# Autodesk Inventor assembly: Arm 2.0 Assembly
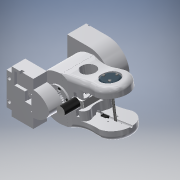
[picture p0: Inventor's stored thumbnail of the model, 180x180]
Saved by Autodesk Inventor 2017 (Build 210142000, 142)
## iProperties
Created: 2017-09-28
Part Number: Arm 2.0 Assembly
Document SubType Name: Assembly
Designer: Zach
Author: Zach
## Documents named in this file (28)
- C:\Users\Dell\Documents\GitHub\tr1\src\Body\Arm Assembly\Shoulder Assembly\Shoulder Assembly, Left.iam
- C:\Users\Dell\Documents\GitHub\tr1\src\Body\Arm Assembly\Shoulder Assembly\Steel Rod 8mm x 135mm.ipt
- C:\Users\Dell\Documents\GitHub\tr1\lib\22x8x8mm Bearing.ipt
- C:\Users\Dell\Documents\GitHub\tr1\src\Body\Arm Assembly\Shoulder Assembly\AA004.ipt
- C:\Users\Dell\Documents\GitHub\tr1\lib\QS12MM250\QS12MM250.ipt
- C:\Users\Dell\Documents\GitHub\tr1\src\Body\Arm Assembly\Shoulder Assembly\AA013.ipt
- C:\Users\Dell\Documents\GitHub\tr1\lib\12V DC Motor 378-1.ipt
- C:\Users\Dell\Documents\GitHub\tr1\lib\Content Center Files\R2017\en-US\ISO 4017(1)\ISO 4017 - M5 x 20 - ISO.ipt
- C:\Users\Dell\Documents\GitHub\tr1\lib\8mm Hub.ipt
- C:\Users\Dell\Documents\GitHub\tr1\src\Body\Arm Assembly\Arm Assembly\Design Accelerator\Spur Gears5.iam
- C:\Users\Dell\Documents\GitHub\tr1\lib\4mm mounting hub.ipt
- C:\Users\Dell\Documents\GitHub\tr1\lib\6201RS\6201RS.ipt
- C:\Users\Dell\Documents\GitHub\tr1\lib\U51105\U51105.ipt
- C:\Users\Dell\Documents\GitHub\tr1\src\Body\Arm Assembly\Shoulder Assembly\AA005b.ipt
- C:\Users\Dell\Documents\GitHub\tr1\src\Body\Arm Assembly\Shoulder Assembly\AA006b.ipt
- C:\Users\Dell\Documents\GitHub\tr1\src\Body\Arm Assembly\Arm Assembly\Design Accelerator\Spur Gears8.iam
- C:\Users\Dell\Documents\GitHub\tr1\src\Body\Arm Assembly\Arm Assembly\Design Accelerator\Spur Gears11.iam
- C:\Users\Dell\Documents\GitHub\tr1\lib\Content Center Files\R2017\en-US\ISO 7045  H\ISO 7045 - M3 x 8 - 4.8 - H - ISO.ipt
- C:\Users\Dell\Documents\GitHub\tr1\lib\Content Center Files\R2017\en-US\ISO 4018\ISO 4018 - M5 x 25.ipt
- C:\Users\Dell\Documents\GitHub\tr1\lib\Content Center Files\R2017\en-US\ISO 7045  H\ISO 7045 - M3 x 12 - 4.8 - H - ISO.ipt
- C:\Users\Dell\Documents\GitHub\tr1\lib\Content Center Files\R2017\en-US\ISO 4762(2)\ISO 4762 - M4 x 10ISO.ipt
- C:\Users\Dell\Documents\GitHub\tr1\lib\6mm Mounting Hub.ipt
- C:\Users\Dell\Documents\GitHub\tr1\lib\TSINY TS-42GZ495.ipt
- C:\Users\Dell\Documents\GitHub\tr1\lib\EMS22XXX-D28-LSX.ipt
- C:\Users\Dell\Documents\GitHub\tr1\src\Body\Arm Assembly\Shoulder Assembly\AA053.ipt
- C:\Users\Dell\Documents\GitHub\tr1\src\Body\Arm Assembly\Shoulder Assembly\AA057.ipt
- C:\Users\Dell\Documents\GitHub\tr1\src\Body\Arm Assembly\Shoulder Assembly\AASG02a.ipt
- C:\Users\Dell\Documents\GitHub\tr1\src\Body\Arm Assembly\Shoulder Assembly\AA001l.ipt
## Components (63 placed, 27 different names)
1. AA001l:1 — Mate:1312, Mate:1313, Mate:1314, Mate:1316, Mate:1317, Mate:1319, Mate:1320, Mate:1321, Mate:1322, Mate:1323, Mate:1324, Mate:1325, Mate:1326, Mate:1327, Mate:1328, Mate:1331, Mate:1332, Angle:18
2. AA004:1 — Mate:23, Mate:345, Mate:347, Mate:350, Mate:357, Mate:590
3. AA005b:1 — Mate:537, Mate:538, Mate:539, Mate:541, Mate:542, Mate:543, Mate:806, Mate:807, Mate:808, Mate:809, Mate:838, Mate:909, Mate:910
4. AA006b:1 — Mate:594, Mate:598, Mate:599, Mate:609, Mate:802, Mate:803, Mate:804, Mate:805, Mate:838, Mate:1088, Mate:1089, Angle:17, Mate:1233
5. AA013:2 — Mate:142, Mate:143, Mate:144, Mate:145, Mate:146, Mate:147, Mate:1281, Mate:1317, Mate:1318
6. AA053:3 — Mate:1331, Mate:1332, Angle:18
7. AA057:1 — Mate:1293, Mate:1295, Mate:1296, Mate:1297, Mate:1323
8. 22x8x8mm Bearing:1 — Mate:433, Mate:1316, Mate:1318
9. 22x8x8mm Bearing:2 — Mate:437
10. QS12MM250:1 — Mate:23, Mate:344, Mate:346, Mate:348, Mate:354, Mate:537, Mate:594, Mate:597, Mate:1230
11. Steel Rod 8mm x 140mm:1 — Mate:433, Mate:437, Mate:575, Flush:35
12. TSINY TS-42GZ495:1 — Mate:1293, Mate:1324, Mate:1325, Mate:1326, Mate:1329, Mate:1330
13. 12V DC Motor 378-1:6 — Mate:340, Mate:342, Mate:538, Mate:539, Mate:540, Mate:543, Mate:907, Mate:908
14. 6201RS:1 — Mate:346, Mate:347
15. 6201RS:2 — Mate:357, Mate:597
16. U51105:1 — Mate:348, Mate:349, Mate:542
17. U51105:2 — Mate:354, Mate:608, Mate:609, Mate:600
18. 6mm Mounting Hub:5 — Mate:1177, Mate:1178, Mate:1179, Mate:1300, Mate:1301, Mate:1302, Mate:1303, Mate:1304, Mate:1305
19. 6mm Mounting Hub:2 — Mate:1090, Mate:1091
20. 8mm Hub:4 — Mate:580, Mate:582, Flush:35, Mate:1315
21. 4mm mounting hub:1 — Mate:340, Mate:540, Mate:541, Mate:887
22. EMS22XXX-D28-LSX:1 — Mate:1088, Mate:1089, Angle:17, Mate:1090, Mate:1091, Mate:1182, Mate:1232
23. EMS22XXX-D28-LSX:2 — Mate:1177, Mate:1180, Mate:1319, Mate:1320
24. AASG01 [sub-assembly] — Mate:342, Mate:344, Mate:345, Mate:349, Mate:350, Mate:810, Mate:811, Mate:812, Mate:813, Mate:814, Mate:815, Mate:816, Mate:817, Mate:818, Mate:819, Mate:820, Mate:821, Mate:887, Mate:888, Mate:889, Mate:890, Mate:891, Mate:1314
25. AASG02a — Mate:1295, Mate:1296, Mate:1297, Mate:1306, Mate:1307, Mate:1308, Mate:1309, Mate:1310, Mate:1311
26. AASG04 [sub-assembly] — Mate:575, Mate:580, Mate:582, Mate:917, Mate:918, Mate:919, Mate:920, Mate:921, Mate:922, Mate:1178, Mate:1179, Mate:1180, Mate:1315, Mate:1321, Mate:1322
27. AASG05 [sub-assembly] — Mate:590, Mate:608, Mate:827, Mate:828, Mate:829, Mate:830, Mate:831, Mate:832, Mate:833, Mate:1182, Mate:1230, Mate:1232, Mate:1233
28. ISO 7045 H M3 x 8 - 4.8 - H:16 — Mate:908, Mate:910
29. ISO 7045 H M3 x 8 - 4.8 - H:17 — Mate:907, Mate:909
30. ISO 7045 H M3 x 12 - 4.8 - H:8 — Mate:889, Mate:890
31. ISO 7045 H M3 x 12 - 4.8 - H:9 — Mate:888, Mate:891
32. ISO 7045 H M3 x 12 - 4.8 - H:13 — Mate:919, Mate:920
33. ISO 7045 H M3 x 12 - 4.8 - H:14 — Mate:917, Mate:921
34. ISO 7045 H M3 x 12 - 4.8 - H:15 — Mate:918, Mate:922
35. ISO 4762 M4 x 10:1 — Mate:1327, Mate:1330
36. ISO 4762 M4 x 10:2 — Mate:1328, Mate:1329
37. ISO 4017 M5 x 20:1 — Mate:146, Mate:147, Mate:1281
38. ISO 4017 M5 x 20:2 — Mate:144, Mate:145
39. ISO 4017 M5 x 20:3 — Mate:142, Mate:143
40. ISO 4018 M5 x 25:7 — Mate:802, Mate:803
41. ISO 4018 M5 x 25:8 — Mate:804, Mate:805
42. ISO 4018 M5 x 25:9 — Mate:806, Mate:808
43. ISO 4018 M5 x 25:10 — Mate:807, Mate:809
44. ISO 4018 M5 x 25:11 — Mate:812, Mate:820
45. ISO 4018 M5 x 25:12 — Mate:810, Mate:816, Mate:1312
46. ISO 4018 M5 x 25:13 — Mate:811, Mate:821, Mate:1313
47. ISO 4018 M5 x 25:14 — Mate:814, Mate:817
48. ISO 4018 M5 x 25:15 — Mate:813, Mate:819
49. ISO 4018 M5 x 25:16 — Mate:815, Mate:818
50. ISO 4018 M5 x 25:17 — Mate:831
51. ISO 4018 M5 x 25:18 — Mate:829
52. ISO 4018 M5 x 25:19 — Mate:832
53. ISO 4018 M5 x 25:20 — Mate:827, Mate:828
54. ISO 4018 M5 x 25:21 — Mate:833
55. ISO 4018 M5 x 25:22 — Mate:830
56. ISO 4018 M5 x 25:23
57. ISO 4018 M5 x 25:24
58. ISO 7045 H M3 x 12 - 4.8 - H:16 — Mate:1300, Mate:1301
59. ISO 7045 H M3 x 12 - 4.8 - H:17 — Mate:1303, Mate:1305
60. ISO 7045 H M3 x 12 - 4.8 - H:18 — Mate:1302, Mate:1304
61. ISO 4017 M5 x 20:4 — Mate:1306, Mate:1310
62. ISO 4017 M5 x 20:5 — Mate:1307, Mate:1309
63. ISO 4017 M5 x 20:6 — Mate:1308, Mate:1311
## Relationships (134: Mate 131, Angle 2, Flush 1)
- Mate:23: AA004:1 ↔ QS12MM250:1
- Mate:142: AA013:2 ↔ ISO 4017 M5 x 20:3
- Mate:143: AA013:2 ↔ ISO 4017 M5 x 20:3
- Mate:144: AA013:2 ↔ ISO 4017 M5 x 20:2
- Mate:145: AA013:2 ↔ ISO 4017 M5 x 20:2
- Mate:146: AA013:2 ↔ ISO 4017 M5 x 20:1
- Mate:147: AA013:2 ↔ ISO 4017 M5 x 20:1
- Mate:340: 12V DC Motor 378-1:6 ↔ 4mm mounting hub:1
- Mate:342: 12V DC Motor 378-1:6 ↔ AASG01
- Mate:344: QS12MM250:1 ↔ AASG01
- Mate:345: AA004:1 ↔ AASG01
- Mate:346: QS12MM250:1 ↔ 6201RS:1
- Mate:347: AA004:1 ↔ 6201RS:1
- Mate:348: QS12MM250:1 ↔ U51105:1
- Mate:349: U51105:1 ↔ AASG01
- Mate:350: AA004:1 ↔ AASG01
- Mate:354: QS12MM250:1 ↔ U51105:2
- Mate:357: AA004:1 ↔ 6201RS:2
- Mate:433: 22x8x8mm Bearing:1 ↔ Steel Rod 8mm x 140mm:1
- Mate:437: 22x8x8mm Bearing:2 ↔ Steel Rod 8mm x 140mm:1
- Mate:537: AA005b:1 ↔ QS12MM250:1
- Mate:538: AA005b:1 ↔ 12V DC Motor 378-1:6
- Mate:539: AA005b:1 ↔ 12V DC Motor 378-1:6
- Mate:540: 12V DC Motor 378-1:6 ↔ 4mm mounting hub:1
- Mate:541: AA005b:1 ↔ 4mm mounting hub:1
- Mate:542: AA005b:1 ↔ U51105:1
- Mate:543: AA005b:1 ↔ 12V DC Motor 378-1:6
- Mate:575: Steel Rod 8mm x 140mm:1 ↔ AASG04
- Mate:580: 8mm Hub:4 ↔ AASG04
- Mate:582: 8mm Hub:4 ↔ AASG04
- Mate:590: AA004:1 ↔ AASG05
- Mate:594: AA006b:1 ↔ QS12MM250:1
- Mate:597: QS12MM250:1 ↔ 6201RS:2
- Mate:598: AA006b:1
- Mate:599: AA006b:1
- Mate:600: U51105:2
- Mate:608: U51105:2 ↔ AASG05
- Mate:609: AA006b:1 ↔ U51105:2
- Mate:802: AA006b:1 ↔ ISO 4018 M5 x 25:7
- Mate:803: AA006b:1 ↔ ISO 4018 M5 x 25:7
- Mate:804: AA006b:1 ↔ ISO 4018 M5 x 25:8
- Mate:805: AA006b:1 ↔ ISO 4018 M5 x 25:8
- Mate:806: AA005b:1 ↔ ISO 4018 M5 x 25:9
- Mate:807: AA005b:1 ↔ ISO 4018 M5 x 25:10
- Mate:808: AA005b:1 ↔ ISO 4018 M5 x 25:9
- Mate:809: AA005b:1 ↔ ISO 4018 M5 x 25:10
- Mate:810: AASG01 ↔ ISO 4018 M5 x 25:12
- Mate:811: AASG01 ↔ ISO 4018 M5 x 25:13
- Mate:812: AASG01 ↔ ISO 4018 M5 x 25:11
- Mate:813: AASG01 ↔ ISO 4018 M5 x 25:15
- Mate:814: AASG01 ↔ ISO 4018 M5 x 25:14
- Mate:815: AASG01 ↔ ISO 4018 M5 x 25:16
- Mate:816: AASG01 ↔ ISO 4018 M5 x 25:12
- Mate:817: AASG01 ↔ ISO 4018 M5 x 25:14
- Mate:818: AASG01 ↔ ISO 4018 M5 x 25:16
- Mate:819: AASG01 ↔ ISO 4018 M5 x 25:15
- Mate:820: AASG01 ↔ ISO 4018 M5 x 25:11
- Mate:821: AASG01 ↔ ISO 4018 M5 x 25:13
- Mate:827: AASG05 ↔ ISO 4018 M5 x 25:20
- Mate:828: AASG05 ↔ ISO 4018 M5 x 25:20
- Mate:829: AASG05 ↔ ISO 4018 M5 x 25:18
- Mate:830: AASG05 ↔ ISO 4018 M5 x 25:22
- Mate:831: AASG05 ↔ ISO 4018 M5 x 25:17
- Mate:832: AASG05 ↔ ISO 4018 M5 x 25:19
- Mate:833: AASG05 ↔ ISO 4018 M5 x 25:21
- Mate:838: AA005b:1 ↔ AA006b:1
- Mate:887: 4mm mounting hub:1 ↔ AASG01
- Mate:888: AASG01 ↔ ISO 7045 H M3 x 12 - 4.8 - H:9
- Mate:889: AASG01 ↔ ISO 7045 H M3 x 12 - 4.8 - H:8
- Mate:890: AASG01 ↔ ISO 7045 H M3 x 12 - 4.8 - H:8
- Mate:891: AASG01 ↔ ISO 7045 H M3 x 12 - 4.8 - H:9
- Mate:907: 12V DC Motor 378-1:6 ↔ ISO 7045 H M3 x 8 - 4.8 - H:17
- Mate:908: 12V DC Motor 378-1:6 ↔ ISO 7045 H M3 x 8 - 4.8 - H:16
- Mate:909: AA005b:1 ↔ ISO 7045 H M3 x 8 - 4.8 - H:17
- Mate:910: AA005b:1 ↔ ISO 7045 H M3 x 8 - 4.8 - H:16
- Mate:917: AASG04 ↔ ISO 7045 H M3 x 12 - 4.8 - H:14
- Mate:918: AASG04 ↔ ISO 7045 H M3 x 12 - 4.8 - H:15
- Mate:919: AASG04 ↔ ISO 7045 H M3 x 12 - 4.8 - H:13
- Mate:920: AASG04 ↔ ISO 7045 H M3 x 12 - 4.8 - H:13
- Mate:921: AASG04 ↔ ISO 7045 H M3 x 12 - 4.8 - H:14
- Mate:922: AASG04 ↔ ISO 7045 H M3 x 12 - 4.8 - H:15
- Mate:1088: AA006b:1 ↔ EMS22XXX-D28-LSX:1
- Mate:1089: AA006b:1 ↔ EMS22XXX-D28-LSX:1
- Angle:17 (90 deg): AA006b:1 ↔ EMS22XXX-D28-LSX:1
- Mate:1090: 6mm Mounting Hub:2 ↔ EMS22XXX-D28-LSX:1
- Mate:1091: 6mm Mounting Hub:2 ↔ EMS22XXX-D28-LSX:1
- Flush:35: Steel Rod 8mm x 140mm:1 ↔ 8mm Hub:4
- Mate:1177: 6mm Mounting Hub:5 ↔ EMS22XXX-D28-LSX:2
- Mate:1178: 6mm Mounting Hub:5 ↔ AASG04
- Mate:1179: 6mm Mounting Hub:5 ↔ AASG04
- Mate:1180: EMS22XXX-D28-LSX:2 ↔ AASG04
- Mate:1182: EMS22XXX-D28-LSX:1 ↔ AASG05
- Mate:1230: QS12MM250:1 ↔ AASG05
- Mate:1232: EMS22XXX-D28-LSX:1 ↔ AASG05
- Mate:1233: AA006b:1 ↔ AASG05
- Mate:1281: AA013:2 ↔ ISO 4017 M5 x 20:1
- Mate:1293: AA057:1 ↔ TSINY TS-42GZ495:1
- Mate:1295: AA057:1 ↔ AASG02a
- Mate:1296: AA057:1 ↔ AASG02a
- Mate:1297: AA057:1 ↔ AASG02a
- Mate:1300: 6mm Mounting Hub:5 ↔ ISO 7045 H M3 x 12 - 4.8 - H:16
- Mate:1301: 6mm Mounting Hub:5 ↔ ISO 7045 H M3 x 12 - 4.8 - H:16
- Mate:1302: 6mm Mounting Hub:5 ↔ ISO 7045 H M3 x 12 - 4.8 - H:18
- Mate:1303: 6mm Mounting Hub:5 ↔ ISO 7045 H M3 x 12 - 4.8 - H:17
- Mate:1304: 6mm Mounting Hub:5 ↔ ISO 7045 H M3 x 12 - 4.8 - H:18
- Mate:1305: 6mm Mounting Hub:5 ↔ ISO 7045 H M3 x 12 - 4.8 - H:17
- Mate:1306: AASG02a ↔ ISO 4017 M5 x 20:4
- Mate:1307: AASG02a ↔ ISO 4017 M5 x 20:5
- Mate:1308: AASG02a ↔ ISO 4017 M5 x 20:6
- Mate:1309: AASG02a ↔ ISO 4017 M5 x 20:5
- Mate:1310: AASG02a ↔ ISO 4017 M5 x 20:4
- Mate:1311: AASG02a ↔ ISO 4017 M5 x 20:6
- Mate:1312: AA001l:1 ↔ ISO 4018 M5 x 25:12
- Mate:1313: AA001l:1 ↔ ISO 4018 M5 x 25:13
- Mate:1314: AA001l:1 ↔ AASG01
- Mate:1315: 8mm Hub:4 ↔ AASG04
- Mate:1316: AA001l:1 ↔ 22x8x8mm Bearing:1
- Mate:1317: AA001l:1 ↔ AA013:2
- Mate:1318: AA013:2 ↔ 22x8x8mm Bearing:1
- Mate:1319: AA001l:1 ↔ EMS22XXX-D28-LSX:2
- Mate:1320: AA001l:1 ↔ EMS22XXX-D28-LSX:2
- Mate:1321: AA001l:1 ↔ AASG04
- Mate:1322: AA001l:1 ↔ AASG04
- Mate:1323: AA001l:1 ↔ AA057:1
- Mate:1324: AA001l:1 ↔ TSINY TS-42GZ495:1
- Mate:1325: AA001l:1 ↔ TSINY TS-42GZ495:1
- Mate:1326: AA001l:1 ↔ TSINY TS-42GZ495:1
- Mate:1327: AA001l:1 ↔ ISO 4762 M4 x 10:1
- Mate:1328: AA001l:1 ↔ ISO 4762 M4 x 10:2
- Mate:1329: TSINY TS-42GZ495:1 ↔ ISO 4762 M4 x 10:2
- Mate:1330: TSINY TS-42GZ495:1 ↔ ISO 4762 M4 x 10:1
- Mate:1331: AA001l:1 ↔ AA053:3
- Mate:1332: AA001l:1 ↔ AA053:3
- Angle:18 (180 deg): AA001l:1 ↔ AA053:3
